# Autodesk Inventor assembly: BearingHousing
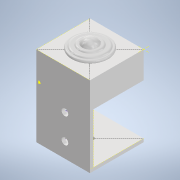
[picture p0: Inventor's stored thumbnail of the model, 180x180]
Saved by Autodesk Inventor 2020 (Build 240168000, 168)
## iProperties
Created: 2021-12-14
Part Number: BearingHousing
Document SubType Name: Assembly
Designer: danie
Author: danie
## Documents named in this file (3)
- C:\Users\danie\Documents\Capstone\Solidworks\BearingHousing.iam
- C:\Users\danie\Documents\Capstone\Solidworks\Bearing Housing.ipt
- C:\Users\danie\Downloads\6421K41_Press-Fit Ball Transfer.ipt
## Components (2 placed, 2 different names)
1. Bearing Housing:1 — Rotational:1
2. 6421K41_Press-Fit Ball Transfer:1 — Rotational:1
## Relationships (1: RevoluteJoint 1)
- Rotational:1 [RevoluteJoint]: Bearing Housing:1 ↔ 6421K41_Press-Fit Ball Transfer:1
